# Autodesk Inventor assembly: 12-16 Frame
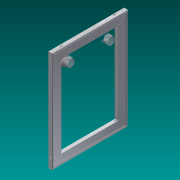
[picture p0: Inventor's stored thumbnail of the model, 180x180]
Saved by Autodesk Inventor 2013 (Build 170138000, 138)
## iProperties
Created: 2013-08-15
Part Number: 12-16 Frame
Document SubType Name: Assembly
Designer: Sawaiz
Author: Sawaiz
## Documents named in this file (6)
- S:\Sawaiz\Documents\3D Modeling\Inventor\PolarGraph\12-16 Frame.iam
- S:\Sawaiz\Documents\3D Modeling\Inventor\PolarGraph\Stretcher\Stretcher-12.ipt
- S:\Sawaiz\Documents\3D Modeling\Inventor\PolarGraph\Stretcher.ipt
- S:\Sawaiz\Documents\3D Modeling\Inventor\PolarGraph\Stretcher\Stretcher-16.ipt
- S:\Sawaiz\Documents\3D Modeling\Inventor\Twitter Flip V 1\Stepper Motor 28BYJ-48.ipt
- S:\Sawaiz\Documents\3D Modeling\Inventor\PolarGraph\MonoFilamentSpool.ipt
## Components (7 placed, 4 different names)
1. Stretcher-12:1 — Mate:1, Mate:2, Mate:4, Mate:5, Mate:7, Mate:8
2. Stretcher-12:2 — Mate:3, Mate:6
3. Stretcher-16:3 — Mate:2, Mate:5
4. Stretcher-16:4 — Mate:1, Mate:3, Mate:4, Mate:6
5. Stepper Motor 28BYJ-48:1 — Mate:8
6. Stepper Motor 28BYJ-48:2 — Mate:7, Flush:1
7. MonoFilamentSpool:1 — Flush:1
## Relationships (9: Mate 8, Flush 1)
- Mate:1: Stretcher-12:1 ↔ Stretcher-16:4
- Mate:2: Stretcher-12:1 ↔ Stretcher-16:3
- Mate:3: Stretcher-12:2 ↔ Stretcher-16:4
- Mate:4: Stretcher-12:1 ↔ Stretcher-16:4
- Mate:5: Stretcher-12:1 ↔ Stretcher-16:3
- Mate:6: Stretcher-12:2 ↔ Stretcher-16:4
- Mate:7: Stretcher-12:1 ↔ Stepper Motor 28BYJ-48:2
- Mate:8: Stretcher-12:1 ↔ Stepper Motor 28BYJ-48:1
- Flush:1: Stepper Motor 28BYJ-48:2 ↔ MonoFilamentSpool:1
